# Autodesk Inventor assembly: MG-Chip Schaufel
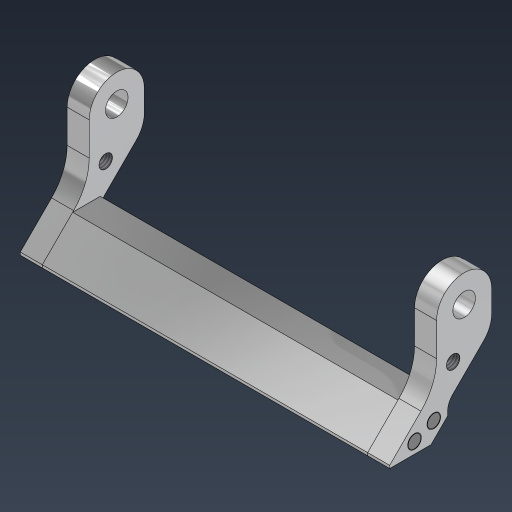
[picture p0: Inventor's stored thumbnail of the model, 512x512]
Saved by Autodesk Inventor 2023.1 (Build 271208000, 208)
## iProperties
Part Number: MG-Chip Schaufel
Material: Generisch
Document SubType Name: Assembly
Designer: rYan
Mass: 11.9053 g
Surface Area: 38.0629 cm^2
Volume: 4.02651 cm^3
Density: 2.95673 g/cm^3
Author: rYan
## Documents named in this file (4)
- D:\TIGERsGIT\Hardware\mechanik\2024\Inventor\Robot\Kicker\MG-Chip Schaufel.iam
- D:\TIGERsGIT\Hardware\mechanik\2024\Inventor\Robot\Kicker\Chip Schaufel Mitte.ipt
- D:\TIGERsGIT\Hardware\mechanik\2024\Inventor\Robot\Kicker\Chip Schaufel Seite.ipt
- D:\TIGERsGIT\Hardware\mechanik\2024\Inventor\Inhaltscenter\de-DE\ISO 2338(2)\ISO 2338 - 2,5 m6 x 10.ipt
## Components (7 placed, 3 different names)
1. Chip Schaufel Mitte:1 — Einfügen:5, Einfügen:6, Passend:1, Passend:2, Fluchtend:1, Fluchtend:2, Fluchtend:3
2. Chip Schaufel Seite:1 — Einfügen:2, Einfügen:3, Einfügen:5, Passend:1
3. Chip Schaufel Seite:2 — Einfügen:1, Einfügen:4, Einfügen:6, Passend:2
4. ISO 2338 2,5 m6 x 10:2 — Einfügen:2
5. ISO 2338 2,5 m6 x 10:1 — Einfügen:1
6. ISO 2338 2,5 m6 x 10:3 — Einfügen:3
7. ISO 2338 2,5 m6 x 10:4 — Einfügen:4
## Relationships (11: Insert 6, Flush 3, Mate 2)
- Einfügen:1 [Insert]: Chip Schaufel Seite:2 ↔ ISO 2338 2,5 m6 x 10:1
- Einfügen:2 [Insert]: Chip Schaufel Seite:1 ↔ ISO 2338 2,5 m6 x 10:2
- Einfügen:3 [Insert]: Chip Schaufel Seite:1 ↔ ISO 2338 2,5 m6 x 10:3
- Einfügen:4 [Insert]: Chip Schaufel Seite:2 ↔ ISO 2338 2,5 m6 x 10:4
- Einfügen:5 [Insert]: Chip Schaufel Mitte:1 ↔ Chip Schaufel Seite:1
- Einfügen:6 [Insert]: Chip Schaufel Mitte:1 ↔ Chip Schaufel Seite:2
- Passend:1 [Mate]: Chip Schaufel Mitte:1 ↔ Chip Schaufel Seite:1
- Passend:2 [Mate]: Chip Schaufel Mitte:1 ↔ Chip Schaufel Seite:2
- Fluchtend:1 [Flush]: Chip Schaufel Mitte:1
- Fluchtend:2 [Flush]: Chip Schaufel Mitte:1
- Fluchtend:3 [Flush]: Chip Schaufel Mitte:1
